# Autodesk Inventor assembly: Lidar Sensor Assembly
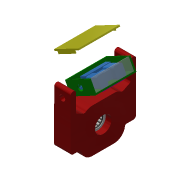
[picture p0: Inventor's stored thumbnail of the model, 180x180]
Saved by Autodesk Inventor 2018.3 (Build 223284000, 284)
## iProperties
Created: 2018-12-21
Part Number: Lidar Sensor Assembly
Document SubType Name: Assembly
Designer: aye06091
Mass: 83.3293 g
Surface Area: 347.329 cm^2
Volume: 82.7348 cm^3
Density: 1.00719 g/cm^3
Author: aye06091
## Documents named in this file (4)
- Y:\DeSimony-R\Senior R&D\4 R&D Shared Folder\VisiStick\VisiStick (Inventor)\Physical Parts\Lidar Sensor Assembly.iam
- Y:\DeSimony-R\Senior R&D\4 R&D Shared Folder\VisiStick\VisiStick (Inventor)\Physical Parts\Needle Bearing.ipt
- Y:\DeSimony-R\Senior R&D\4 R&D Shared Folder\VisiStick\VisiStick (Inventor)\Physical Parts\Needle Bearing Mount.ipt
- Y:\DeSimony-R\Senior R&D\4 R&D Shared Folder\VisiStick\VisiStick (Inventor)\Physical Parts\Sharp 2Y0A02 Assembled Case.iam
## Components (3 placed, 3 different names)
1. Needle Bearing:1 — Insert:1
2. Needle Bearing Mount:1 — Insert:1, Cylindrical:1, Mate:1
3. Sharp 2Y0A02 Assembled Case:1 [sub-assembly] — Cylindrical:1, Mate:1
## Relationships (3: Insert 1, CylindricalJoint 1, Mate 1)
- Insert:1: Needle Bearing:1 ↔ Needle Bearing Mount:1
- Cylindrical:1: Needle Bearing Mount:1 ↔ Sharp 2Y0A02 Assembled Case:1
- Mate:1 (1.27 mm): Needle Bearing Mount:1 ↔ Sharp 2Y0A02 Assembled Case:1
